# Autodesk Inventor assembly: BAcA_assembly
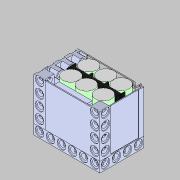
[picture p0: Inventor's stored thumbnail of the model, 180x180]
Saved by Autodesk Inventor 2019.3 (Build 233278000, 278)
## iProperties
Created: 2019-02-15
Part Number: BAcA_assembly
Document SubType Name: Assembly
Designer: Varga Daniel
Sending System: SolidWorks 2018
Last Author: david
Last Saved: 2019-02-15
Author: Varga Daniel
## Documents named in this file (6)
- C:\!_Dani\!_cloud\OneDrive\!_munka\Revolution\RevvyDemoKit\Structural parts\Demo parts\Battery\Inventor Imported\BAcA_assembly.iam
- C:\!_Dani\!_cloud\OneDrive\!_munka\Revolution\RevvyDemoKit\Structural parts\Demo parts\Battery\Inventor Imported\BAcA.ipt
- C:\!_Dani\!_cloud\OneDrive\!_munka\Revolution\RevvyDemoKit\Structural parts\Demo parts\Battery\Inventor Imported\BAcA_2.ipt
- C:\!_Dani\!_cloud\OneDrive\!_munka\Revolution\RevvyDemoKit\Structural parts\Demo parts\Battery\Inventor Imported\Battery_holder_WZY-148-1_with_cable.iam
- C:\!_Dani\!_cloud\OneDrive\!_munka\Revolution\RevvyDemoKit\Structural parts\Connetor Pins\CP1+x1+\CP1x1.ipt
- C:\!_Dani\!_cloud\OneDrive\!_munka\Revolution\RevvyDemoKit\Structural parts\Demo parts\Battery\Inventor Imported\BAcA_3.ipt
## Components (122 placed, 5 different names)
1. BAcA:1 — Flush:1, Mate:1, Mate:2, Mate:3, Tangent:1, Angle:1, Insert:1, Insert:2, Insert:3, Insert:4, Insert:5, Insert:6, Insert:7, Insert:8, Insert:9, Insert:10, Insert:11, Insert:12, Insert:13, Angle:2, Mate:4, Flush:2, Flush:3
2. BAcA_2:1 — Flush:1, Mate:1, Mate:2
3. Battery_holder_WZY-148-1_with_cable:1 [sub-assembly] — Mate:3, Tangent:1, Angle:1, Tangent:2, Mate:4
4. CP1x1:99 — Insert:11
5. CP1x1:100 — Insert:12
6. CP1x1:101 — Insert:13
7. CP1x1:96 — Insert:8
8. BAcA_3:1 — Flush:2, Flush:3
9. CP1x1:1 — Insert:1
10. CP1x1:2
11. CP1x1:3
12. CP1x1:4
13. CP1x1:5
14. CP1x1:6
15. CP1x1:7
16. CP1x1:8
17. CP1x1:9
18. CP1x1:10
19. CP1x1:11
20. CP1x1:12
21. CP1x1:13
22. CP1x1:14
23. CP1x1:15
24. CP1x1:16
25. CP1x1:17
26. CP1x1:18
27. CP1x1:19
28. CP1x1:20
29. CP1x1:21
30. CP1x1:22
31. CP1x1:23
32. CP1x1:24
33. CP1x1:25
34. CP1x1:26
35. CP1x1:27
36. CP1x1:28
37. CP1x1:29
38. CP1x1:30
39. CP1x1:31
40. CP1x1:32
41. CP1x1:33 — Insert:2
42. CP1x1:34
43. CP1x1:35
44. CP1x1:36
45. CP1x1:37
46. CP1x1:38
47. CP1x1:39
48. CP1x1:40
49. CP1x1:41
50. CP1x1:42
51. CP1x1:43
52. CP1x1:44
53. CP1x1:45
54. CP1x1:46
55. CP1x1:47
56. CP1x1:48
57. CP1x1:49
58. CP1x1:50
59. CP1x1:51
60. CP1x1:52
61. CP1x1:53
62. CP1x1:54
63. CP1x1:55
64. CP1x1:56
65. CP1x1:57 — Insert:3
66. CP1x1:58
67. CP1x1:59
68. CP1x1:60
69. CP1x1:61
70. CP1x1:62
71. CP1x1:63
72. CP1x1:64
73. CP1x1:65
74. CP1x1:66
75. CP1x1:67
76. CP1x1:68
77. CP1x1:69
78. CP1x1:70
79. CP1x1:71
80. CP1x1:72
81. CP1x1:73
82. CP1x1:74
83. CP1x1:75
84. CP1x1:76
85. CP1x1:77
86. CP1x1:78
87. CP1x1:79
88. CP1x1:80
89. CP1x1:81 — Insert:4
90. CP1x1:82
91. CP1x1:83
92. CP1x1:84
93. CP1x1:85 — Insert:5
94. CP1x1:86
95. CP1x1:87
96. CP1x1:88
97. CP1x1:89
98. CP1x1:90
99. CP1x1:91 — Insert:6
100. CP1x1:92
101. CP1x1:93
102. CP1x1:94
103. CP1x1:98 — Insert:10
104. CP1x1:102
105. CP1x1:103
106. CP1x1:104
107. CP1x1:105
108. CP1x1:106
109. CP1x1:97 — Insert:9
110. CP1x1:107
111. CP1x1:108
112. CP1x1:109
113. CP1x1:110
114. CP1x1:111
115. CP1x1:112
116. CP1x1:95 — Insert:7
117. CP1x1:113
118. CP1x1:114
119. CP1x1:115
120. CP1x1:116
121. CP1x1:117
122. CP1x1:118
## Component patterns: (32 elements, first: CP1x1:1), (24 elements, first: CP1x1:33), (24 elements, first: CP1x1:57), (4 elements, first: CP1x1:81), (6 elements, first: CP1x1:85), (4 elements, first: CP1x1:91), (6 elements, first: CP1x1:98), (7 elements, first: CP1x1:97), (7 elements, first: CP1x1:95)
## Relationships (24: Insert 13, Mate 4, Flush 3, Tangent 2, Angle 2)
- Flush:1: BAcA:1 ↔ BAcA_2:1
- Mate:1: BAcA:1 ↔ BAcA_2:1
- Mate:2: BAcA:1 ↔ BAcA_2:1
- Mate:3: BAcA:1 ↔ Battery_holder_WZY-148-1_with_cable:1
- Tangent:1: BAcA:1 ↔ Battery_holder_WZY-148-1_with_cable:1
- Angle:1 (180 deg): BAcA:1 ↔ Battery_holder_WZY-148-1_with_cable:1
- Insert:1: BAcA:1 ↔ CP1x1:1
- Insert:2: BAcA:1 ↔ CP1x1:33
- Insert:3: BAcA:1 ↔ CP1x1:57
- Insert:4: BAcA:1 ↔ CP1x1:81
- Insert:5: BAcA:1 ↔ CP1x1:85
- Insert:6: BAcA:1 ↔ CP1x1:91
- Insert:7: BAcA:1 ↔ CP1x1:95
- Insert:8: BAcA:1 ↔ CP1x1:96
- Insert:9: BAcA:1 ↔ CP1x1:97
- Insert:10: BAcA:1 ↔ CP1x1:98
- Insert:11: BAcA:1 ↔ CP1x1:99
- Insert:12: BAcA:1 ↔ CP1x1:100
- Insert:13: BAcA:1 ↔ CP1x1:101
- Angle:2 (0 deg): BAcA:1
- Tangent:2: Battery_holder_WZY-148-1_with_cable:1
- Mate:4 (3.678 mm): BAcA:1 ↔ Battery_holder_WZY-148-1_with_cable:1
- Flush:2: BAcA:1 ↔ BAcA_3:1
- Flush:3: BAcA:1 ↔ BAcA_3:1
